# Autodesk Inventor assembly: Knee_MIR
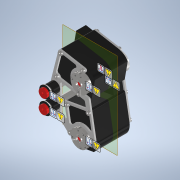
[picture p0: Inventor's stored thumbnail of the model, 180x180]
Saved by Autodesk Inventor 2020.4 (Build 244396000, 396)
## iProperties
Created: 2021-09-06
Part Number: Knee_MIR
Document SubType Name: Assembly
Designer: Masato Kubotera
Mass: 264.861 g
Surface Area: 473.637 cm^2
Volume: 130.531 cm^3
Density: 2.0291 g/cm^3
Author: Masato
## Documents named in this file (17)
- C:\Users\Masato\Documents\Inventor\CIT Brains_Inventor\OpenPlatform_ver3_0\LowerBody\Knee\Knee_MIR.iam
- C:\Users\Masato\Documents\Inventor\CIT Brains_Inventor\OpenPlatform_ver3_0\LowerBody\Knee\Knee_side_frame.ipt
- C:\Users\Masato\Documents\Inventor\CIT Brains_Inventor\OpenPlatform_ver3_0\ReadyMade\KONDO\B3M-SC-1170-A.ipt
- C:\Users\Masato\Documents\Inventor\CIT Brains_Inventor\OpenPlatform_ver3_0\ReadyMade\KONDO\ClampHorn.ipt
- C:\Users\Masato\Documents\Inventor\CIT Brains_Inventor\OpenPlatform_ver3_0\ReadyMade\KONDO\FreeHorn.ipt
- C:\Users\Masato\Documents\Inventor\CIT Brains_Inventor\OpenPlatform_ver3_0\ReadyMade\Bush\80F-0603.ipt
- C:\Users\Masato\Documents\Inventor\CIT Brains_Inventor\OpenPlatform_ver3_0\ReadyMade\Washer\UUW-0412-10BH.ipt
- C:\Users\Masato\Documents\Inventor\CIT Brains_Inventor\OpenPlatform_ver3_0\ReadyMade\Washer\CC-0612-15B.ipt
- C:\Users\Masato\Documents\Inventor\CIT Brains_Inventor\OpenPlatform_ver3_0\ReadyMade\Washer\CC-0612-50B.ipt
- C:\Users\Masato\Documents\Inventor\CIT Brains_Inventor\OpenPlatform_ver3_0\ReadyMade\Spacer\SLSBF6-39.5-M4-N4.ipt
- C:\Users\Masato\Documents\Inventor\CIT Brains_Inventor\OpenPlatform_ver3_0\ReadyMade\Screw\DBTS4-11-8.ipt
- C:\Users\Masato\Documents\Inventor\CIT Brains_Inventor\OpenPlatform_ver3_0\ReadyMade\Washer\UUW-0614-05BH.ipt
- C:\Users\Masato\Documents\Inventor\CIT Brains_Inventor\OpenPlatform_ver3_0\ReadyMade\Washer\TT-0814-10.ipt
- C:\Users\Masato\Documents\Inventor\CIT Brains_Inventor\OpenPlatform_ver3_0\ReadyMade\KONDO\FreeHorn_Screw.ipt
- C:\Users\Masato\Documents\Inventor\CIT Brains_Inventor\OpenPlatform_ver3_0\ReadyMade\Screw\620103008.ipt
- C:\Users\Masato\Documents\Inventor\CIT Brains_Inventor\OpenPlatform_ver3_0\ReadyMade\Screw\M2_6-15.ipt
- C:\Users\Masato\Documents\Inventor\CIT Brains_Inventor\OpenPlatform_ver3_0\ReadyMade\Screw\M2_6-20.ipt
## Components (58 placed, 16 different names)
1. Knee_side_frame:1 — フラッシュ:1, メイト:2, メイト:1, 挿入:6, 挿入:5, 挿入:8, 挿入:7, 挿入:3, 挿入:4, 挿入:1, 挿入:2, 挿入:9, 挿入:10, 挿入:12, 挿入:11, 挿入:13, 挿入:14, 挿入:15, 挿入:16, 角度:1, 挿入:33, 挿入:34, 挿入:37, 挿入:38
2. Knee_side_frame:2 — 挿入:22, 挿入:24, 挿入:21, 挿入:23, 挿入:20, 挿入:19, 挿入:18, 挿入:17, 挿入:26, 挿入:25, 挿入:28, 挿入:27, 挿入:31, 挿入:30, 挿入:32, 挿入:29, 挿入:35, 挿入:36, 挿入:39, 挿入:40
3. B3M-SC-1170-A:1 — 挿入:20, 挿入:19, 挿入:3, 挿入:4, 挿入:18, 挿入:17, 挿入:1, 挿入:2, 挿入:61, 挿入:63, 挿入:59, 挿入:57, 角度:3
4. B3M-SC-1170-A:2 — 挿入:6, 挿入:22, 挿入:24, 挿入:21, 挿入:23, 挿入:5, 挿入:8, 挿入:7, 挿入:62, 挿入:64, 挿入:60, 挿入:58, 角度:4
5. ClampHorn:1 — 挿入:57, フラッシュ:2, 角度:3
6. ClampHorn:2 — 挿入:58, フラッシュ:3, 角度:4
7. FreeHorn:1 — 挿入:61, フラッシュ:2
8. FreeHorn:2 — 挿入:62, フラッシュ:3
9. 80F-0603:1 — 挿入:49
10. 80F-0603:2 — 挿入:50
11. 80F-0603:3 — 挿入:51
12. 80F-0603:4 — 挿入:52
13. UUW-0412-10BH:1 — 挿入:41, 挿入:37, 挿入:136
14. UUW-0412-10BH:2 — 挿入:38, 挿入:42, 挿入:135
15. UUW-0412-10BH:3 — 挿入:43, 挿入:39, 挿入:137
16. UUW-0412-10BH:4 — 挿入:40, 挿入:44, 挿入:138
17. CC-0612-15B:1 — 挿入:45, 挿入:41
18. CC-0612-15B:2 — 挿入:46, 挿入:42
19. CC-0612-15B:3 — 挿入:47, 挿入:43
20. CC-0612-15B:4 — 挿入:48, 挿入:44
21. CC-0612-50B:1 — 挿入:49, 挿入:45
22. CC-0612-50B:2 — 挿入:50, 挿入:46
23. CC-0612-50B:3 — 挿入:51, 挿入:47
24. CC-0612-50B:4 — 挿入:52, 挿入:48
25. SLSBF6-39.5-M4-N4:1 — 角度:1, 挿入:35, 挿入:33, 角度:2
26. SLSBF6-39.5-M4-N4:2 — 角度:2, 挿入:36, 挿入:34
27. DBTS4-11-8:1 — 挿入:138, 挿入:142
28. DBTS4-11-8:2 — 挿入:137, 挿入:141
29. DBTS4-11-8:3 — 挿入:135, 挿入:139
30. DBTS4-11-8:4 — 挿入:136, 挿入:140
31. UUW-0614-05BH:1 — 挿入:141, 挿入:145
32. UUW-0614-05BH:2 — 挿入:139, 挿入:144
33. UUW-0614-05BH:3 — 挿入:140, 挿入:143
34. UUW-0614-05BH:4 — 挿入:142, 挿入:146
35. TT-0814-10:1 — 挿入:143
36. TT-0814-10:2 — 挿入:144
37. TT-0814-10:3 — 挿入:146
38. TT-0814-10:4 — 挿入:145
39. FreeHorn_Screw:1 — 挿入:63
40. FreeHorn_Screw:2 — 挿入:64
41. 620103008:1 — 挿入:59
42. 620103008:2 — 挿入:60
43. M2_6-15:1 — 挿入:9
44. M2_6-15:2 — 挿入:10
45. M2_6-15:3 — 挿入:11
46. M2_6-15:4 — 挿入:12
47. M2_6-15:5 — 挿入:13
48. M2_6-15:6 — 挿入:14
49. M2_6-15:7 — 挿入:15
50. M2_6-15:8 — 挿入:16
51. M2_6-20:1 — 挿入:25
52. M2_6-20:2 — 挿入:26
53. M2_6-20:3 — 挿入:27
54. M2_6-20:4 — 挿入:28
55. M2_6-20:5 — 挿入:29
56. M2_6-20:6 — 挿入:30
57. M2_6-20:7 — 挿入:31
58. M2_6-20:8 — 挿入:32
## Relationships (81: Insert 72, Angle 4, Flush 3, Mate 2)
- フラッシュ:1 [Flush]: Knee_side_frame:1
- メイト:2 [Mate] (19.75 mm): Knee_side_frame:1
- メイト:1 [Mate]: Knee_side_frame:1
- 挿入:6 [Insert]: Knee_side_frame:1 ↔ B3M-SC-1170-A:2
- 挿入:22 [Insert]: Knee_side_frame:2 ↔ B3M-SC-1170-A:2
- 挿入:24 [Insert]: Knee_side_frame:2 ↔ B3M-SC-1170-A:2
- 挿入:21 [Insert]: Knee_side_frame:2 ↔ B3M-SC-1170-A:2
- 挿入:23 [Insert]: Knee_side_frame:2 ↔ B3M-SC-1170-A:2
- 挿入:5 [Insert]: Knee_side_frame:1 ↔ B3M-SC-1170-A:2
- 挿入:8 [Insert]: Knee_side_frame:1 ↔ B3M-SC-1170-A:2
- 挿入:7 [Insert]: Knee_side_frame:1 ↔ B3M-SC-1170-A:2
- 挿入:20 [Insert]: Knee_side_frame:2 ↔ B3M-SC-1170-A:1
- 挿入:19 [Insert]: Knee_side_frame:2 ↔ B3M-SC-1170-A:1
- 挿入:3 [Insert]: Knee_side_frame:1 ↔ B3M-SC-1170-A:1
- 挿入:4 [Insert]: Knee_side_frame:1 ↔ B3M-SC-1170-A:1
- 挿入:18 [Insert]: Knee_side_frame:2 ↔ B3M-SC-1170-A:1
- 挿入:17 [Insert]: Knee_side_frame:2 ↔ B3M-SC-1170-A:1
- 挿入:1 [Insert]: Knee_side_frame:1 ↔ B3M-SC-1170-A:1
- 挿入:2 [Insert]: Knee_side_frame:1 ↔ B3M-SC-1170-A:1
- 挿入:62 [Insert]: B3M-SC-1170-A:2 ↔ FreeHorn:2
- 挿入:61 [Insert]: B3M-SC-1170-A:1 ↔ FreeHorn:1
- 挿入:9 [Insert]: Knee_side_frame:1 ↔ M2_6-15:1
- 挿入:10 [Insert]: Knee_side_frame:1 ↔ M2_6-15:2
- 挿入:12 [Insert]: Knee_side_frame:1 ↔ M2_6-15:4
- 挿入:11 [Insert]: Knee_side_frame:1 ↔ M2_6-15:3
- 挿入:13 [Insert]: Knee_side_frame:1 ↔ M2_6-15:5
- 挿入:14 [Insert]: Knee_side_frame:1 ↔ M2_6-15:6
- 挿入:15 [Insert]: Knee_side_frame:1 ↔ M2_6-15:7
- 挿入:16 [Insert]: Knee_side_frame:1 ↔ M2_6-15:8
- 挿入:26 [Insert]: Knee_side_frame:2 ↔ M2_6-20:2
- 挿入:25 [Insert]: Knee_side_frame:2 ↔ M2_6-20:1
- 挿入:28 [Insert]: Knee_side_frame:2 ↔ M2_6-20:4
- 挿入:27 [Insert]: Knee_side_frame:2 ↔ M2_6-20:3
- 挿入:31 [Insert]: Knee_side_frame:2 ↔ M2_6-20:7
- 挿入:30 [Insert]: Knee_side_frame:2 ↔ M2_6-20:6
- 挿入:32 [Insert]: Knee_side_frame:2 ↔ M2_6-20:8
- 挿入:29 [Insert]: Knee_side_frame:2 ↔ M2_6-20:5
- 挿入:50 [Insert]: 80F-0603:2 ↔ CC-0612-50B:2
- 挿入:46 [Insert]: CC-0612-15B:2 ↔ CC-0612-50B:2
- 挿入:49 [Insert]: 80F-0603:1 ↔ CC-0612-50B:1
- 挿入:45 [Insert]: CC-0612-15B:1 ↔ CC-0612-50B:1
- 挿入:51 [Insert]: 80F-0603:3 ↔ CC-0612-50B:3
- 挿入:47 [Insert]: CC-0612-15B:3 ↔ CC-0612-50B:3
- 挿入:52 [Insert]: 80F-0603:4 ↔ CC-0612-50B:4
- 挿入:48 [Insert]: CC-0612-15B:4 ↔ CC-0612-50B:4
- 挿入:64 [Insert]: B3M-SC-1170-A:2 ↔ FreeHorn_Screw:2
- 挿入:63 [Insert]: B3M-SC-1170-A:1 ↔ FreeHorn_Screw:1
- 角度:1 [Angle] (0 deg): Knee_side_frame:1 ↔ SLSBF6-39.5-M4-N4:1
- 挿入:35 [Insert]: Knee_side_frame:2 ↔ SLSBF6-39.5-M4-N4:1
- 挿入:33 [Insert]: Knee_side_frame:1 ↔ SLSBF6-39.5-M4-N4:1
- 角度:2 [Angle] (0 deg): SLSBF6-39.5-M4-N4:1 ↔ SLSBF6-39.5-M4-N4:2
- 挿入:36 [Insert]: Knee_side_frame:2 ↔ SLSBF6-39.5-M4-N4:2
- 挿入:34 [Insert]: Knee_side_frame:1 ↔ SLSBF6-39.5-M4-N4:2
- 挿入:41 [Insert]: UUW-0412-10BH:1 ↔ CC-0612-15B:1
- 挿入:37 [Insert]: Knee_side_frame:1 ↔ UUW-0412-10BH:1
- 挿入:38 [Insert]: Knee_side_frame:1 ↔ UUW-0412-10BH:2
- 挿入:42 [Insert]: UUW-0412-10BH:2 ↔ CC-0612-15B:2
- 挿入:43 [Insert]: UUW-0412-10BH:3 ↔ CC-0612-15B:3
- 挿入:39 [Insert]: Knee_side_frame:2 ↔ UUW-0412-10BH:3
- 挿入:40 [Insert]: Knee_side_frame:2 ↔ UUW-0412-10BH:4
- 挿入:44 [Insert]: UUW-0412-10BH:4 ↔ CC-0612-15B:4
- 挿入:59 [Insert]: B3M-SC-1170-A:1 ↔ 620103008:1
- 挿入:60 [Insert]: B3M-SC-1170-A:2 ↔ 620103008:2
- 挿入:58 [Insert]: B3M-SC-1170-A:2 ↔ ClampHorn:2
- フラッシュ:3 [Flush]: ClampHorn:2 ↔ FreeHorn:2
- 角度:4 [Angle] (0 deg): B3M-SC-1170-A:2 ↔ ClampHorn:2
- 挿入:57 [Insert]: B3M-SC-1170-A:1 ↔ ClampHorn:1
- フラッシュ:2 [Flush]: ClampHorn:1 ↔ FreeHorn:1
- 角度:3 [Angle] (0 deg): B3M-SC-1170-A:1 ↔ ClampHorn:1
- 挿入:138 [Insert]: UUW-0412-10BH:4 ↔ DBTS4-11-8:1
- 挿入:137 [Insert]: UUW-0412-10BH:3 ↔ DBTS4-11-8:2
- 挿入:135 [Insert]: UUW-0412-10BH:2 ↔ DBTS4-11-8:3
- 挿入:136 [Insert]: UUW-0412-10BH:1 ↔ DBTS4-11-8:4
- 挿入:141 [Insert]: DBTS4-11-8:2 ↔ UUW-0614-05BH:1
- 挿入:139 [Insert]: DBTS4-11-8:3 ↔ UUW-0614-05BH:2
- 挿入:140 [Insert]: DBTS4-11-8:4 ↔ UUW-0614-05BH:3
- 挿入:142 [Insert]: DBTS4-11-8:1 ↔ UUW-0614-05BH:4
- 挿入:143 [Insert]: UUW-0614-05BH:3 ↔ TT-0814-10:1
- 挿入:144 [Insert]: UUW-0614-05BH:2 ↔ TT-0814-10:2
- 挿入:146 [Insert]: UUW-0614-05BH:4 ↔ TT-0814-10:3
- 挿入:145 [Insert]: UUW-0614-05BH:1 ↔ TT-0814-10:4
